# Autodesk Inventor assembly: Earbud Assembly
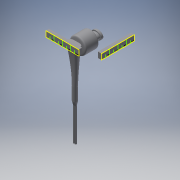
[picture p0: Inventor's stored thumbnail of the model, 180x180]
Saved by Autodesk Inventor 2016 (Build 200138000, 138)
## iProperties
Created: 2015-08-01
Part Number: Earbud Assembly
Document SubType Name: Assembly
Designer: Nancy
Author: Nancy
## Documents named in this file (4)
- C:\Users\Nancy\Documents\Inventor Files\Earbud Assembly.iam
- C:\Users\Nancy\Documents\Inventor Files\Earbud Casing\Earbud Casing.ipt
- C:\Users\Nancy\Documents\Inventor Files\Male End AJ.ipt
- C:\Users\Nancy\Documents\Inventor Files\1 inch Ruler.ipt
## Components (4 placed, 3 different names)
1. Earbud Casing:1 — Insert:1
2. Male End AJ:1 — Insert:1
3. 1 inch Ruler:1
4. 1 inch Ruler:2
## Relationships (1: Insert 1)
- Insert:1 (-15 mm): Earbud Casing:1 ↔ Male End AJ:1
